# Autodesk Inventor assembly: 3DoF Manipulator Type 2
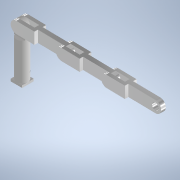
[picture p0: Inventor's stored thumbnail of the model, 180x180]
Saved by Autodesk Inventor 2021 (Build 250183000, 183)
## iProperties
Created: 2023-06-27
Part Number: 3DoF Manipulator Type 2
Document SubType Name: Assembly
Designer: fist5
Mass: 3515.18 g
Surface Area: 2009.55 cm^2
Volume: 1301.92 cm^3
Density: 2.7 g/cm^3
Author: fist5
## Documents named in this file (4)
- C:\Users\fist5\Desktop\3DoF Manipulator Type 2.iam
- C:\Users\fist5\Desktop\Manipulator Base Type2.ipt
- C:\Users\fist5\Desktop\Manipulator Link Type 2.ipt
- C:\Users\fist5\Desktop\Manipulator Link Type 1.ipt
## Components (5 placed, 3 different names)
1. Manipulator Base Type2:1 — Mate:1, Mate:2
2. Manipulator Link Type 2:1 — Mate:1, Mate:2, Mate:3, Mate:4
3. Manipulator Link Type 1:1 — Mate:3, Mate:4, Mate:5, Mate:6
4. Manipulator Link Type 1:2 — Mate:5, Mate:6, Mate:7, Mate:8
5. Manipulator Link Type 1:3 — Mate:7, Mate:8
## Relationships (8: Mate 8)
- Mate:1: Manipulator Base Type2:1 ↔ Manipulator Link Type 2:1
- Mate:2: Manipulator Base Type2:1 ↔ Manipulator Link Type 2:1
- Mate:3: Manipulator Link Type 2:1 ↔ Manipulator Link Type 1:1
- Mate:4: Manipulator Link Type 2:1 ↔ Manipulator Link Type 1:1
- Mate:5: Manipulator Link Type 1:1 ↔ Manipulator Link Type 1:2
- Mate:6: Manipulator Link Type 1:1 ↔ Manipulator Link Type 1:2
- Mate:7: Manipulator Link Type 1:2 ↔ Manipulator Link Type 1:3
- Mate:8: Manipulator Link Type 1:2 ↔ Manipulator Link Type 1:3
